# Autodesk Inventor assembly: ADSK-MH-10024
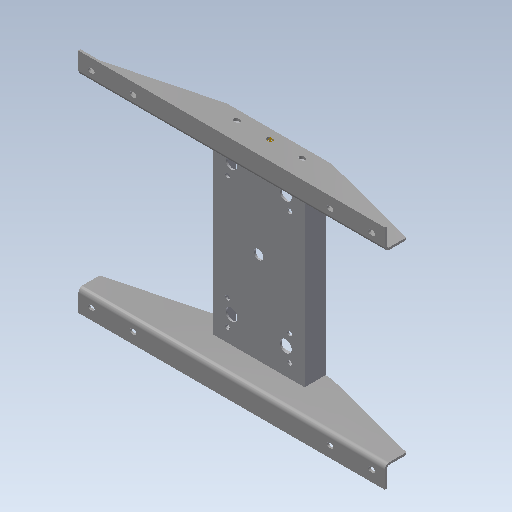
[picture p0: Inventor's stored thumbnail of the model, 512x512]
Saved by Autodesk Inventor 2020.2 (Build 242310000, 310)
## iProperties
Created: 2008-03-10
Part Number: ADSK-MH-10024
Document SubType Name: Assembly
Designer: R.O'mahony
Description: Pnematic Support Beam
Engineer: Demir Ali
Checked By: Demir Ali
Company: Autodesk Ltd
Author: R.O'mahony
Keywords: Roller Conveyor
Revision Number: A
## Documents named in this file (3)
- C:\Users\peter\source\repos\InventorDA-FLC\Dataset\Discharge Conveyor\ADSK-MH-10024.iam
- C:\Users\peter\source\repos\InventorDA-FLC\Dataset\Discharge Conveyor\ADSK-MH-10025.ipt
- C:\Users\peter\source\repos\InventorDA-FLC\Dataset\Discharge Conveyor\ADSK-MH-10026.ipt
## Components (3 placed, 3 different names)
1. ADSK-MH-10025:2 — Mate:1, Angle:1, Mate:2
2. Discharge_cross_member — Mate:1, Angle:1, Mate:2
3. ADSK-MH-10026:2
## Component patterns: (2 elements, first: Discharge_cross_member)
## Relationships (3: Mate 2, Angle 1)
- Mate:1: ADSK-MH-10025:2 ↔ Discharge_cross_member
- Angle:1 (0 deg): ADSK-MH-10025:2 ↔ Discharge_cross_member
- Mate:2: ADSK-MH-10025:2 ↔ Discharge_cross_member
